# Autodesk Inventor assembly: CNC-Y-axis- ASSEMBLYg
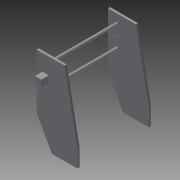
[picture p0: Inventor's stored thumbnail of the model, 180x180]
Saved by Autodesk Inventor 2015 (Build 190159000, 159)
## iProperties
Created: 2015-03-24
Part Number: CNC-Y-axis- ASSEMBLYg
Document SubType Name: Assembly
Designer: Bangladesh
Author: Bangladesh
## Documents named in this file (5)
- C:\Users\Alvi\Documents\CNC design files\Assemblies\CNC-Y-axis- ASSEMBLY.iam
- C:\Users\Alvi\Documents\CNC design files\CNC-Y-axis- side plates.ipt
- C:\Users\Alvi\Documents\CNC design files\CNC-Y-axs- sliding rod.ipt
- C:\Users\Alvi\Documents\CNC design files\CNC-Y-axis- side plates with stepper.ipt
- C:\Users\Alvi\Documents\CNC design files\CNC- Stepper Motor.ipt
## Components (5 placed, 4 different names)
1. CNC-Y-axis- side plates:1 — Mate:1, Mate:2
2. CNC-Y-axs- sliding rod:1 — Mate:1, Mate:3
3. CNC-Y-axs- sliding rod:2 — Mate:2, Mate:4
4. CNC-Y-axis- side plates with stepper:1 — Mate:3, Mate:4, Mate:5, Mate:6
5. CNC- Stepper Motor:1 — Mate:5, Mate:6
## Relationships (6: Mate 6)
- Mate:1: CNC-Y-axis- side plates:1 ↔ CNC-Y-axs- sliding rod:1
- Mate:2: CNC-Y-axis- side plates:1 ↔ CNC-Y-axs- sliding rod:2
- Mate:3: CNC-Y-axs- sliding rod:1 ↔ CNC-Y-axis- side plates with stepper:1
- Mate:4: CNC-Y-axs- sliding rod:2 ↔ CNC-Y-axis- side plates with stepper:1
- Mate:5: CNC-Y-axis- side plates with stepper:1 ↔ CNC- Stepper Motor:1
- Mate:6: CNC-Y-axis- side plates with stepper:1 ↔ CNC- Stepper Motor:1
